# Autodesk Inventor assembly: NASA-20-HUB
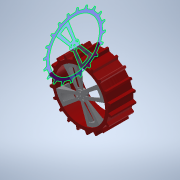
[picture p0: Inventor's stored thumbnail of the model, 180x180]
Saved by Autodesk Inventor 2020 (Build 240168000, 168)
## iProperties
Created: 2019-09-21
Part Number: NASA-20-HUB
Document SubType Name: Assembly
Designer: Rick Szalay
Author: Rick Szalay
## Documents named in this file (6)
- C:\Users\Rick Szalay\Documents\NASA-20\NASA-20\HUB\NASA-20-HUB.iam
- C:\Users\Rick Szalay\Documents\NASA-20\NASA-20\HUB\9604T110_FLANGE-MOUNT SHAFT COLLAR.ipt
- C:\Users\Rick Szalay\Documents\NASA-20\NASA-20\HUB\NASA-20-HUB-SPK-01.ipt
- C:\Users\Rick Szalay\Documents\Inventor\Content Center Files\R2020\en-US\DIN 912\DIN 912 - M3 x 0.5 x 20 x 18.75.ipt
- C:\Users\Rick Szalay\Documents\NASA-20\NASA-20\HUB\NASA-20-TRD-01.ipt
- C:\Users\Rick Szalay\Documents\NASA-20\NASA-20\HUB\NASA-20-SHFT-01.ipt
## Components (8 placed, 5 different names)
1. 9604T110_FLANGE-MOUNT SHAFT COLLAR:1 — Mate:1, Flush:1, Flush:2, Mate:5, Mate:6, Mate:7
2. NASA-20-HUB-SPK-01:1 — Mate:2, Mate:3, Mate:4, Mate:6, Mate:7, Insert:1, Insert:2, Insert:3, Mate:8, Flush:3, Mate:10
3. NASA-20-HUB-SPK-01:2 — Mate:2, Mate:3, Mate:4, Mate:5, Mate:9
4. DIN 912 - replaced by DIN EN ISO 4762 M3 x 20:1 — Insert:1
5. DIN 912 - replaced by DIN EN ISO 4762 M3 x 20:2 — Insert:2
6. DIN 912 - replaced by DIN EN ISO 4762 M3 x 20:3 — Insert:3
7. NASA-20-TRD-01:1 — Mate:8, Flush:3
8. NASA-20-SHFT-01:1 — Mate:9, Mate:10
## Relationships (16: Mate 10, Flush 3, Insert 3)
- Mate:1: 9604T110_FLANGE-MOUNT SHAFT COLLAR:1
- Flush:1: 9604T110_FLANGE-MOUNT SHAFT COLLAR:1
- Flush:2: 9604T110_FLANGE-MOUNT SHAFT COLLAR:1
- Mate:2: NASA-20-HUB-SPK-01:1 ↔ NASA-20-HUB-SPK-01:2
- Mate:3: NASA-20-HUB-SPK-01:1 ↔ NASA-20-HUB-SPK-01:2
- Mate:4: NASA-20-HUB-SPK-01:1 ↔ NASA-20-HUB-SPK-01:2
- Mate:5: 9604T110_FLANGE-MOUNT SHAFT COLLAR:1 ↔ NASA-20-HUB-SPK-01:2
- Mate:6: 9604T110_FLANGE-MOUNT SHAFT COLLAR:1 ↔ NASA-20-HUB-SPK-01:1
- Mate:7: 9604T110_FLANGE-MOUNT SHAFT COLLAR:1 ↔ NASA-20-HUB-SPK-01:1
- Insert:1: NASA-20-HUB-SPK-01:1 ↔ DIN 912 - replaced by DIN EN ISO 4762 M3 x 20:1
- Insert:2: NASA-20-HUB-SPK-01:1 ↔ DIN 912 - replaced by DIN EN ISO 4762 M3 x 20:2
- Insert:3: NASA-20-HUB-SPK-01:1 ↔ DIN 912 - replaced by DIN EN ISO 4762 M3 x 20:3
- Mate:8: NASA-20-HUB-SPK-01:1 ↔ NASA-20-TRD-01:1
- Flush:3 (17.5006 mm): NASA-20-HUB-SPK-01:1 ↔ NASA-20-TRD-01:1
- Mate:9: NASA-20-HUB-SPK-01:2 ↔ NASA-20-SHFT-01:1
- Mate:10: NASA-20-HUB-SPK-01:1 ↔ NASA-20-SHFT-01:1
